# Autodesk Inventor assembly: Nose assembly
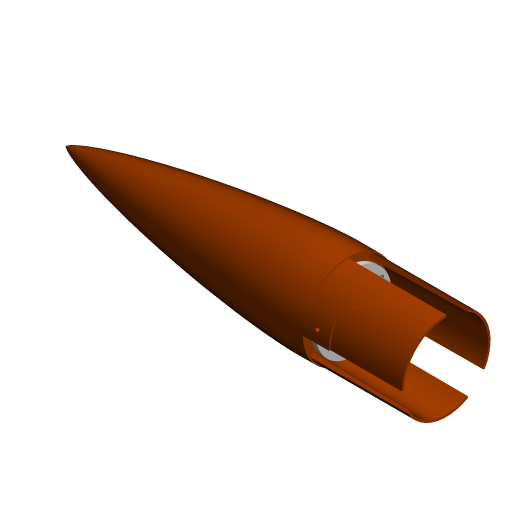
[picture p0: Inventor's stored thumbnail of the model, 512x512]
Saved by Autodesk Inventor 2024 (Build 280153000, 153)
## iProperties
Part Number: Nose assembly
Document SubType Name: Assembly
Designer: Jamie
Author: Jamie
## Documents named in this file (5)
- C:\Users\Jamie\Documents\Uni\DARE\Scrambler-2-CAD\Autodesk\Nose assembly.iam
- C:\Users\Jamie\Documents\Uni\DARE\Scrambler-2-CAD\Autodesk\smoke_grenade.ipt
- C:\Users\Jamie\Documents\Uni\DARE\Scrambler-2-CAD\Autodesk\grenade_retention_ring.ipt
- C:\Users\Jamie\Documents\Uni\DARE\Scrambler-2-CAD\Autodesk\Nosecone base.ipt
- C:\Users\Jamie\Documents\Uni\DARE\Scrambler-2-CAD\Autodesk\Nosecone top.ipt
## Components (4 placed, 4 different names)
1. smoke_grenade:1 — Rotational:1, Mate:3
2. grenade_retention_ring:1 — Rotational:1, Mate:4
3. Nosecone base:1 — Mate:1, Mate:2, Mate:3, Mate:4
4. Nosecone top:1 — Mate:1, Mate:2
## Relationships (5: Mate 4, RevoluteJoint 1)
- Rotational:1 [RevoluteJoint] (5 mm): smoke_grenade:1 ↔ grenade_retention_ring:1
- Mate:1: Nosecone base:1 ↔ Nosecone top:1
- Mate:2: Nosecone base:1 ↔ Nosecone top:1
- Mate:3: smoke_grenade:1 ↔ Nosecone base:1
- Mate:4: grenade_retention_ring:1 ↔ Nosecone base:1
